# Autodesk Inventor assembly: Assembly1
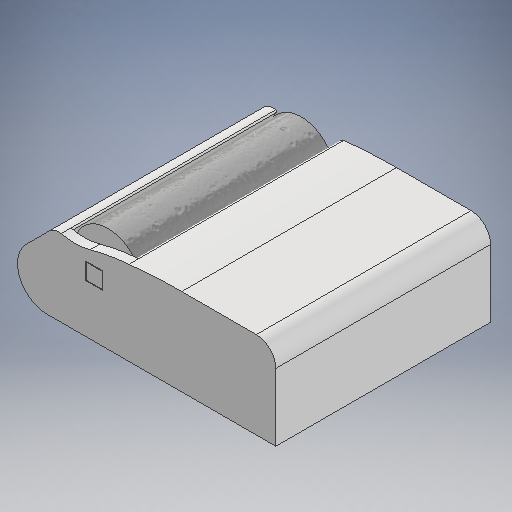
[picture p0: Inventor's stored thumbnail of the model, 512x512]
Saved by Autodesk Inventor 2025.2 (Build 292293000, 293)
## iProperties
Created: 2025-02-14
Part Number: Assembly1
Document SubType Name: Assembly
Designer: Alex
Author: Alex
## Documents named in this file (4)
- C:\Shared\alex-bartella-schoolwork\4b03\a1\Assembly1.iam
- C:\Shared\alex-bartella-schoolwork\4b03\a1\roller.ipt
- C:\Shared\alex-bartella-schoolwork\4b03\a1\tank.ipt
- C:\Shared\alex-bartella-schoolwork\4b03\a1\shaft.ipt
## Components (3 placed, 3 different names)
1. roller:1 — Mate:1
2. tank:1 — Mate:2, Mate:3
3. shaft:1 — Mate:1, Mate:2, Mate:3
## Relationships (3: Mate 3)
- Mate:1: roller:1 ↔ shaft:1
- Mate:2 (0.35 mm): tank:1 ↔ shaft:1
- Mate:3: tank:1 ↔ shaft:1
